# Autodesk Inventor assembly: FullV2
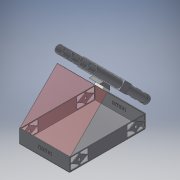
[picture p0: Inventor's stored thumbnail of the model, 180x180]
Saved by Autodesk Inventor 2019 (Build 230136000, 136)
## iProperties
Created: 2021-09-16
Part Number: FullV2
Document SubType Name: Assembly
Designer: timmy
Author: timmy
## Documents named in this file (8)
- S:\Inventor\RoboCatz\T-Shirt\FullV2.iam
- S:\Inventor\RoboCatz\T-Shirt\NamePlateV1.ipt
- S:\Inventor\RoboCatz\T-Shirt\R-O-SideV1.ipt
- S:\Inventor\RoboCatz\T-Shirt\TopV2.ipt
- S:\Inventor\RoboCatz\T-Shirt\Plexi-SideV!.ipt
- S:\Inventor\RoboCatz\T-Shirt\BackV1.ipt
- S:\Inventor\RoboCatz\T-Shirt\LauncherFullV1.iam
- S:\Inventor\RoboCatz\T-Shirt\BottomV1.ipt
## Components (10 placed, 7 different names)
1. NamePlateV1:1 — Mate:1, Flush:2, Flush:3, Flush:4, Flush:5, Flush:6, Flush:14
2. R-O-SideV1:1 — Flush:4, Flush:5, Flush:6, Mate:6, Flush:11, Mate:9, Mate:10
3. NamePlateV1:2 — Flush:7, Flush:8, Flush:9
4. R-O-SideV1:2 — Mate:1, Flush:2, Flush:3, Flush:7, Flush:8, Flush:9, Mate:2, Angle:1, Mate:3, Angle:3, Flush:10, Mate:7, Mate:8, Mate:17, Flush:15
5. Plexi-SideV!:1 — Flush:11, Mate:9, Mate:10, Mate:12
6. Plexi-SideV!:2 — Flush:10, Mate:7, Mate:8, Mate:11, Flush:12, Flush:13
7. TopV2:1 — Mate:11, Flush:12, Mate:13
8. BackV1:1 — Mate:12, Mate:13, Flush:13, Mate:14, Mate:15, Mate:16
9. LauncherFullV1:1 [sub-assembly] — Mate:14, Mate:15, Mate:16
10. BottomV1:1 — Flush:14, Mate:17, Flush:15
## Relationships (32: Mate 15, Flush 14, Angle 3)
- Mate:1: NamePlateV1:1 ↔ R-O-SideV1:2
- Flush:2: NamePlateV1:1 ↔ R-O-SideV1:2
- Flush:3: NamePlateV1:1 ↔ R-O-SideV1:2
- Flush:4: NamePlateV1:1 ↔ R-O-SideV1:1
- Flush:5: NamePlateV1:1 ↔ R-O-SideV1:1
- Flush:6: NamePlateV1:1 ↔ R-O-SideV1:1
- Flush:7: NamePlateV1:2 ↔ R-O-SideV1:2
- Flush:8: NamePlateV1:2 ↔ R-O-SideV1:2
- Flush:9: NamePlateV1:2 ↔ R-O-SideV1:2
- Mate:2: R-O-SideV1:2
- Angle:1 (45 deg): R-O-SideV1:2
- Mate:3: R-O-SideV1:2
- Angle:2 (90 deg)
- Mate:6: R-O-SideV1:1
- Angle:3 (135 deg): R-O-SideV1:2
- Flush:10: R-O-SideV1:2 ↔ Plexi-SideV!:2
- Mate:7: R-O-SideV1:2 ↔ Plexi-SideV!:2
- Mate:8: R-O-SideV1:2 ↔ Plexi-SideV!:2
- Flush:11: R-O-SideV1:1 ↔ Plexi-SideV!:1
- Mate:9: R-O-SideV1:1 ↔ Plexi-SideV!:1
- Mate:10: R-O-SideV1:1 ↔ Plexi-SideV!:1
- Mate:11: Plexi-SideV!:2 ↔ TopV2:1
- Flush:12: Plexi-SideV!:2 ↔ TopV2:1
- Mate:12: Plexi-SideV!:1 ↔ BackV1:1
- Mate:13: TopV2:1 ↔ BackV1:1
- Flush:13: Plexi-SideV!:2 ↔ BackV1:1
- Mate:14: BackV1:1 ↔ LauncherFullV1:1
- Mate:15: BackV1:1 ↔ LauncherFullV1:1
- Mate:16: BackV1:1 ↔ LauncherFullV1:1
- Flush:14: NamePlateV1:1 ↔ BottomV1:1
- Mate:17: R-O-SideV1:2 ↔ BottomV1:1
- Flush:15: R-O-SideV1:2 ↔ BottomV1:1
